# Autodesk Inventor assembly: Practice Robot
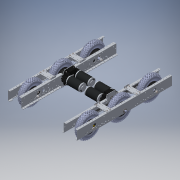
[picture p0: Inventor's stored thumbnail of the model, 180x180]
Saved by Autodesk Inventor 2016 (Build 200138000, 138)
## iProperties
Created: 2017-01-05
Part Number: Practice Robot
Document SubType Name: Assembly
Designer: Dhruv
Author: Dhruv
## Documents named in this file (3)
- C:\Users\Dhruv\Desktop\MISC\FRC 2017\Practice Robot.iam
- C:\Users\Dhruv\Downloads\AM-14U3-PN8+Pneumatic+6WD.iam
- C:\Users\Dhruv\Downloads\am-0255+2.5inch+CIM+Motor.ipt
## Components (5 placed, 2 different names)
1. AM-14U3-PN8+Pneumatic+6WD:1 [sub-assembly] — Insert:1, Insert:2, Insert:3, Insert:4, Insert:5, Insert:6, Insert:7, Insert:8
2. am-0255+2.5inch+CIM+Motor:1 — Insert:3, Insert:4
3. am-0255+2.5inch+CIM+Motor:2 — Insert:7, Insert:8
4. am-0255+2.5inch+CIM+Motor:3 — Insert:5, Insert:6
5. am-0255+2.5inch+CIM+Motor:4 — Insert:1, Insert:2
## Relationships (8: Insert 8)
- Insert:1: AM-14U3-PN8+Pneumatic+6WD:1 ↔ am-0255+2.5inch+CIM+Motor:4
- Insert:2: AM-14U3-PN8+Pneumatic+6WD:1 ↔ am-0255+2.5inch+CIM+Motor:4
- Insert:3: AM-14U3-PN8+Pneumatic+6WD:1 ↔ am-0255+2.5inch+CIM+Motor:1
- Insert:4: AM-14U3-PN8+Pneumatic+6WD:1 ↔ am-0255+2.5inch+CIM+Motor:1
- Insert:5: AM-14U3-PN8+Pneumatic+6WD:1 ↔ am-0255+2.5inch+CIM+Motor:3
- Insert:6: AM-14U3-PN8+Pneumatic+6WD:1 ↔ am-0255+2.5inch+CIM+Motor:3
- Insert:7: AM-14U3-PN8+Pneumatic+6WD:1 ↔ am-0255+2.5inch+CIM+Motor:2
- Insert:8: AM-14U3-PN8+Pneumatic+6WD:1 ↔ am-0255+2.5inch+CIM+Motor:2
